# Autodesk Inventor assembly: Frame_Assembly
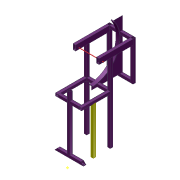
[picture p0: Inventor's stored thumbnail of the model, 180x180]
Saved by Autodesk Inventor 2012 (Build 160160000, 160)
## iProperties
Created: 2012-01-21
Part Number: Frame_Assembly
Document SubType Name: Assembly
Designer: JesseK
Mass: 2937.93 g
Surface Area: 12351.2 cm^2
Volume: 1209.15 cm^3
Density: 2.42974 g/cm^3
Author: JesseK
## Documents named in this file (12)
- Z:\UserData\Documents\Inventor\team1885frc\Robot2012\Conveyor3\Frame_Assembly.iam
- Z:\UserData\Documents\Inventor\team1885frc\Robot2012\Conveyor3\Frame_MainVerticalSupport_Rear.ipt
- Z:\UserData\Documents\Inventor\team1885frc\Robot2012\Conveyor3\Frame_MainShooterFrame_FrontRear.ipt
- Z:\UserData\Documents\Inventor\team1885frc\Robot2012\Conveyor3\Frame_CrossSupport_8in.ipt
- Z:\UserData\Documents\Inventor\team1885frc\Robot2012\Conveyor3\Frame_FrontConveyorGuide.ipt
- Z:\UserData\Documents\Inventor\team1885frc\Robot2012\Conveyor3\Frame_MidFrontRear_Brace.ipt
- Z:\UserData\Documents\Inventor\team1885frc\Robot2012\Conveyor3\Frame_VerticalSideGuide_Long.ipt
- Z:\UserData\Documents\Inventor\team1885frc\Robot2012\Conveyor3\Frame_LowerCrossSupport.ipt
- Z:\UserData\Documents\Inventor\team1885frc\Robot2012\Conveyor3\Frame_FrontConveyorGuideSideSupport.ipt
- Z:\UserData\Documents\Inventor\team1885frc\Robot2012\Conveyor3\Frame_RearVerticalShooterSupport.ipt
- Z:\UserData\Documents\Inventor\team1885frc\Robot2012\Conveyor3\ShooterCurve.ipt
- Z:\UserData\Documents\Inventor\team1885frc\Robot2012\Shooter\CenterFinder.ipt
## Components (18 placed, 11 different names)
1. Frame_MainVerticalSupport_Rear:1 — Mate:5, Mate:24, Flush:16, Mate:41, Mate:57, Flush:22, Mate:72, Flush:30
2. Frame_MainVerticalSupport_Rear:2 — Mate:5, Mate:12, Flush:11, Mate:25, Mate:40, Mate:56
3. Frame_MainShooterFrame_FrontRear:1 — Mate:24, Mate:66, Flush:23, Flush:24, Mate:72, Flush:29, Flush:30
4. Frame_MainShooterFrame_FrontRear:2 — Mate:25, Flush:25, Flush:26, Mate:67, Flush:29, Flush:31
5. Frame_CrossSupport_8in:2 — Mate:12, Flush:11, Flush:13, Flush:14, Mate:57
6. Frame_FrontConveyorGuide:1 — Flush:16, Mate:43, Flush:21, Mate:53, Mate:61, Mate:68
7. Frame_MidFrontRear_Brace:1 — Flush:14, Mate:41, Mate:43, Mate:54
8. Frame_MidFrontRear_Brace:2 — Flush:13, Mate:39, Mate:56, Mate:58, Mate:59, Mate:60
9. Frame_VerticalSideGuide_Long:1 — Mate:39, Mate:40, Mate:54, Flush:22
10. Frame_LowerCrossSupport:1 — Flush:21, Mate:53
11. Frame_FrontConveyorGuideSideSupport:1 — Mate:61, Mate:62, Mate:63, Mate:68
12. Frame_FrontConveyorGuideSideSupport:2 — Mate:58, Mate:59, Mate:60, Mate:62, Mate:63
13. Frame_RearVerticalShooterSupport:1 — Mate:66, Flush:23, Flush:24, Mate:74
14. Frame_RearVerticalShooterSupport:2 — Flush:25, Flush:26, Mate:67, Mate:69, Flush:27, Mate:70, Mate:75, Flush:32, Mate:76
15. Frame_CrossSupport_8in:4 — Mate:69, Flush:27, Mate:70, Mate:71, Flush:28, Mate:74
16. ShooterCurve:1 — Mate:71, Flush:28, Mate:73
17. CenterFinder:1 — Mate:73, Flush:31
18. Frame_CrossSupport_8in:5 — Mate:75, Flush:32, Mate:76
## Relationships (45: Mate 29, Flush 16)
- Mate:5: Frame_MainVerticalSupport_Rear:1 ↔ Frame_MainVerticalSupport_Rear:2
- Mate:12: Frame_MainVerticalSupport_Rear:2 ↔ Frame_CrossSupport_8in:2
- Flush:11: Frame_MainVerticalSupport_Rear:2 ↔ Frame_CrossSupport_8in:2
- Mate:24: Frame_MainVerticalSupport_Rear:1 ↔ Frame_MainShooterFrame_FrontRear:1
- Mate:25: Frame_MainVerticalSupport_Rear:2 ↔ Frame_MainShooterFrame_FrontRear:2
- Flush:13: Frame_CrossSupport_8in:2 ↔ Frame_MidFrontRear_Brace:2
- Flush:14: Frame_CrossSupport_8in:2 ↔ Frame_MidFrontRear_Brace:1
- Flush:16 (25.4 mm): Frame_MainVerticalSupport_Rear:1 ↔ Frame_FrontConveyorGuide:1
- Mate:39: Frame_MidFrontRear_Brace:2 ↔ Frame_VerticalSideGuide_Long:1
- Mate:40 (139.7 mm): Frame_MainVerticalSupport_Rear:2 ↔ Frame_VerticalSideGuide_Long:1
- Mate:41: Frame_MainVerticalSupport_Rear:1 ↔ Frame_MidFrontRear_Brace:1
- Mate:43 (88.9 mm): Frame_FrontConveyorGuide:1 ↔ Frame_MidFrontRear_Brace:1
- Flush:21: Frame_FrontConveyorGuide:1 ↔ Frame_LowerCrossSupport:1
- Mate:53: Frame_FrontConveyorGuide:1 ↔ Frame_LowerCrossSupport:1
- Mate:54: Frame_MidFrontRear_Brace:1 ↔ Frame_VerticalSideGuide_Long:1
- Mate:56: Frame_MainVerticalSupport_Rear:2 ↔ Frame_MidFrontRear_Brace:2
- Mate:57: Frame_MainVerticalSupport_Rear:1 ↔ Frame_CrossSupport_8in:2
- Mate:58: Frame_MidFrontRear_Brace:2 ↔ Frame_FrontConveyorGuideSideSupport:2
- Mate:59: Frame_MidFrontRear_Brace:2 ↔ Frame_FrontConveyorGuideSideSupport:2
- Mate:60: Frame_MidFrontRear_Brace:2 ↔ Frame_FrontConveyorGuideSideSupport:2
- Mate:61: Frame_FrontConveyorGuide:1 ↔ Frame_FrontConveyorGuideSideSupport:1
- Mate:62: Frame_FrontConveyorGuideSideSupport:1 ↔ Frame_FrontConveyorGuideSideSupport:2
- Mate:63: Frame_FrontConveyorGuideSideSupport:1 ↔ Frame_FrontConveyorGuideSideSupport:2
- Flush:22: Frame_MainVerticalSupport_Rear:1 ↔ Frame_VerticalSideGuide_Long:1
- Mate:66: Frame_MainShooterFrame_FrontRear:1 ↔ Frame_RearVerticalShooterSupport:1
- Flush:23: Frame_MainShooterFrame_FrontRear:1 ↔ Frame_RearVerticalShooterSupport:1
- Flush:24: Frame_MainShooterFrame_FrontRear:1 ↔ Frame_RearVerticalShooterSupport:1
- Flush:25: Frame_MainShooterFrame_FrontRear:2 ↔ Frame_RearVerticalShooterSupport:2
- Flush:26: Frame_MainShooterFrame_FrontRear:2 ↔ Frame_RearVerticalShooterSupport:2
- Mate:67: Frame_MainShooterFrame_FrontRear:2 ↔ Frame_RearVerticalShooterSupport:2
- Mate:68: Frame_FrontConveyorGuide:1 ↔ Frame_FrontConveyorGuideSideSupport:1
- Mate:69: Frame_RearVerticalShooterSupport:2 ↔ Frame_CrossSupport_8in:4
- Flush:27: Frame_RearVerticalShooterSupport:2 ↔ Frame_CrossSupport_8in:4
- Mate:70: Frame_RearVerticalShooterSupport:2 ↔ Frame_CrossSupport_8in:4
- Mate:71: Frame_CrossSupport_8in:4 ↔ ShooterCurve:1
- Flush:28: Frame_CrossSupport_8in:4 ↔ ShooterCurve:1
- Mate:72: Frame_MainVerticalSupport_Rear:1 ↔ Frame_MainShooterFrame_FrontRear:1
- Flush:29: Frame_MainShooterFrame_FrontRear:1 ↔ Frame_MainShooterFrame_FrontRear:2
- Flush:30 (-107.95 mm): Frame_MainVerticalSupport_Rear:1 ↔ Frame_MainShooterFrame_FrontRear:1
- Mate:73: ShooterCurve:1 ↔ CenterFinder:1
- Mate:74: Frame_RearVerticalShooterSupport:1 ↔ Frame_CrossSupport_8in:4
- Flush:31 (-12.7 mm): Frame_MainShooterFrame_FrontRear:2 ↔ CenterFinder:1
- Mate:75: Frame_RearVerticalShooterSupport:2 ↔ Frame_CrossSupport_8in:5
- Flush:32: Frame_RearVerticalShooterSupport:2 ↔ Frame_CrossSupport_8in:5
- Mate:76: Frame_RearVerticalShooterSupport:2 ↔ Frame_CrossSupport_8in:5
